# Autodesk Inventor assembly: AgarMouldAssembly
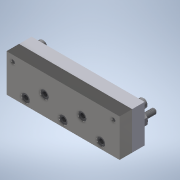
[picture p0: Inventor's stored thumbnail of the model, 180x180]
Saved by Autodesk Inventor 2021 (Build 250183000, 183)
## iProperties
Created: 2016-01-19
Part Number: AgarMouldAssembly
Document SubType Name: Assembly
Designer: 120pa
Author: 120pa
## Documents named in this file (8)
- C:\Users\MicroscopyInnovation\Documents\Inventor\NatProtocolsManuscript\agarose_mould_assembly.iam
- C:\Users\MicroscopyInnovation\Documents\Inventor\NatProtocolsManuscript\agarose_mould_bottom.ipt
- C:\Users\MicroscopyInnovation\Documents\Inventor\NatProtocolsManuscript\agarose_mould.ipt
- C:\Users\MicroscopyInnovation\Documents\Inventor\NatProtocolsManuscript\agarose_holder_peek.ipt
- C:\Users\MicroscopyInnovation\Documents\Inventor\NatProtocolsManuscript\agarose_mould_8_32_screw.ipt
- C:\Users\MicroscopyInnovation\Documents\Inventor\NatProtocolsManuscript\agarose_mould_8_32_nut.ipt
- C:\Users\MicroscopyInnovation\Documents\Inventor\NatProtocolsManuscript\agarose_mould_8_32_screw2.ipt
- C:\Users\MicroscopyInnovation\Documents\Inventor\NatProtocolsManuscript\agarouse_mould_8_32_screw3.ipt
## Components (15 placed, 7 different names)
1. agarose_mould_bottom:1 — Mate:1, Flush:1, Flush:2, Mate:2, Mate:3, Angle:1, Mate:4, Mate:5, Angle:2, Angle:3, Mate:6, Mate:7, Mate:8, Mate:9, Mate:10, Mate:11, Mate:12, Mate:13, Mate:24, Mate:25, Mate:26, Mate:27
2. agarose_mould:1 — Mate:1, Flush:1, Flush:2, Mate:20, Mate:21, Mate:22, Mate:23
3. agarose_holder_peek:1 — Mate:2, Mate:3, Angle:1, Mate:16
4. agarose_holder_peek:2 — Mate:5, Angle:2, Mate:6, Mate:14
5. agarose_holder_peek:3 — Mate:4, Angle:3, Mate:7, Mate:15
6. agarose_mould_8_32_screw:1 — Mate:8, Mate:13, Mate:19
7. agarose_mould_8_32_screw:2 — Mate:9, Mate:12, Mate:17
8. agarose_mould_8_32_screw:3 — Mate:10, Mate:11, Mate:18
9. agarose_mould_8_32_nut:1 — Mate:14, Mate:19
10. agarose_mould_8_32_nut:2 — Mate:15, Mate:17
11. agarose_mould_8_32_nut:3 — Mate:16, Mate:18
12. agarose_mould_8_32_screw2:1 — Mate:20, Mate:23
13. agarose_mould_8_32_screw2:2 — Mate:21, Mate:22
14. agarouse_mould_8_32_screw3:1 — Mate:25, Mate:26
15. agarouse_mould_8_32_screw3:2 — Mate:24, Mate:27
## Relationships (32: Mate 27, Angle 3, Flush 2)
- Mate:1: agarose_mould_bottom:1 ↔ agarose_mould:1
- Flush:1: agarose_mould_bottom:1 ↔ agarose_mould:1
- Flush:2: agarose_mould_bottom:1 ↔ agarose_mould:1
- Mate:2: agarose_mould_bottom:1 ↔ agarose_holder_peek:1
- Mate:3: agarose_mould_bottom:1 ↔ agarose_holder_peek:1
- Angle:1 (180 deg): agarose_mould_bottom:1 ↔ agarose_holder_peek:1
- Mate:4: agarose_mould_bottom:1 ↔ agarose_holder_peek:3
- Mate:5: agarose_mould_bottom:1 ↔ agarose_holder_peek:2
- Angle:2 (0 deg): agarose_mould_bottom:1 ↔ agarose_holder_peek:2
- Angle:3 (0 deg): agarose_mould_bottom:1 ↔ agarose_holder_peek:3
- Mate:6: agarose_mould_bottom:1 ↔ agarose_holder_peek:2
- Mate:7: agarose_mould_bottom:1 ↔ agarose_holder_peek:3
- Mate:8: agarose_mould_bottom:1 ↔ agarose_mould_8_32_screw:1
- Mate:9: agarose_mould_bottom:1 ↔ agarose_mould_8_32_screw:2
- Mate:10: agarose_mould_bottom:1 ↔ agarose_mould_8_32_screw:3
- Mate:11: agarose_mould_bottom:1 ↔ agarose_mould_8_32_screw:3
- Mate:12: agarose_mould_bottom:1 ↔ agarose_mould_8_32_screw:2
- Mate:13: agarose_mould_bottom:1 ↔ agarose_mould_8_32_screw:1
- Mate:14: agarose_holder_peek:2 ↔ agarose_mould_8_32_nut:1
- Mate:15: agarose_holder_peek:3 ↔ agarose_mould_8_32_nut:2
- Mate:16: agarose_holder_peek:1 ↔ agarose_mould_8_32_nut:3
- Mate:17: agarose_mould_8_32_screw:2 ↔ agarose_mould_8_32_nut:2
- Mate:18: agarose_mould_8_32_screw:3 ↔ agarose_mould_8_32_nut:3
- Mate:19: agarose_mould_8_32_screw:1 ↔ agarose_mould_8_32_nut:1
- Mate:20: agarose_mould:1 ↔ agarose_mould_8_32_screw2:1
- Mate:21: agarose_mould:1 ↔ agarose_mould_8_32_screw2:2
- Mate:22: agarose_mould:1 ↔ agarose_mould_8_32_screw2:2
- Mate:23: agarose_mould:1 ↔ agarose_mould_8_32_screw2:1
- Mate:24: agarose_mould_bottom:1 ↔ agarouse_mould_8_32_screw3:2
- Mate:25: agarose_mould_bottom:1 ↔ agarouse_mould_8_32_screw3:1
- Mate:26: agarose_mould_bottom:1 ↔ agarouse_mould_8_32_screw3:1
- Mate:27: agarose_mould_bottom:1 ↔ agarouse_mould_8_32_screw3:2
